# Autodesk Inventor assembly: robot
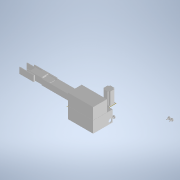
[picture p0: Inventor's stored thumbnail of the model, 180x180]
Saved by Autodesk Inventor 2020 (Build 240168000, 168)
## iProperties
Created: 2021-03-19
Part Number: robot
Document SubType Name: Assembly
Designer: super
Author: super
## Documents named in this file (10)
- C:\desk\promissionsave\inventor\robot\robot.iam
- C:\desk\promissionsave\inventor\robot\corpo.ipt
- C:\desk\promissionsave\inventor\robot\servospt70.ipt
- C:\desk\promissionsave\inventor\robot\balde.ipt
- C:\desk\promissionsave\inventor\robot\armj1.ipt
- C:\desk\promissionsave\inventor\robot\armj2.ipt
- C:\desk\promissionsave\inventor\robot\nema23.ipt
- C:\desk\promissionsave\inventor\robot\armj3.ipt
- C:\desk\promissionsave\inventor\robot\armj4.ipt
- C:\desk\promissionsave\inventor\robot\guia.ipt
## Components (17 placed, 9 different names)
1. corpo:1 — Mate:5, Flush:2, Mate:7, Flush:4, Flush:5, Mate:8, Mate:9, Flush:6, Mate:15, Mate:17, Mate:18, Flush:11
2. servospt70:1 — Mate:8, Mate:9, Flush:6, Rotational:1
3. balde:1 — Mate:7, Flush:4, Flush:5
4. servospt70:2 — Mate:10, Mate:11, Flush:7
5. armj1:1 — Rotational:1, Mate:10, Mate:11, Flush:7, Mate:12, Flush:8, Mate:14, Flush:9
6. armj1:2 — Mate:12, Mate:13, Flush:8
7. armj1:3 — Mate:13
8. armj2:1 — Mate:14, Flush:9, Mate:15, Mate:16, Flush:10
9. armj3:1 — Mate:16, Flush:10, Mate:19
10. servospt70:3
11. nema23:1 — Mate:17, Mate:18, Flush:11
12. armj4:1 — Mate:19
13. guia:1
14. guia:2
15. guia:3
16. guia:4
17. guia:5
## Relationships (24: Mate 14, Flush 9, RevoluteJoint 1)
- Mate:5: corpo:1
- Flush:2: corpo:1
- Mate:7 (1 mm): corpo:1 ↔ balde:1
- Flush:4: corpo:1 ↔ balde:1
- Flush:5: corpo:1 ↔ balde:1
- Mate:8: corpo:1 ↔ servospt70:1
- Mate:9: corpo:1 ↔ servospt70:1
- Flush:6: corpo:1 ↔ servospt70:1
- Rotational:1 [RevoluteJoint]: servospt70:1 ↔ armj1:1
- Mate:10: servospt70:2 ↔ armj1:1
- Mate:11: servospt70:2 ↔ armj1:1
- Flush:7 (10 mm): servospt70:2 ↔ armj1:1
- Mate:12: armj1:1 ↔ armj1:2
- Mate:13: armj1:2 ↔ armj1:3
- Flush:8: armj1:1 ↔ armj1:2
- Mate:14: armj1:1 ↔ armj2:1
- Flush:9: armj1:1 ↔ armj2:1
- Mate:15 (40 mm): corpo:1 ↔ armj2:1
- Mate:16: armj2:1 ↔ armj3:1
- Flush:10: armj2:1 ↔ armj3:1
- Mate:17 (-50 mm): corpo:1 ↔ nema23:1
- Mate:18 (50 mm): corpo:1 ↔ nema23:1
- Flush:11 (81.5 mm): corpo:1 ↔ nema23:1
- Mate:19: armj3:1 ↔ armj4:1
